# Autodesk Inventor assembly: Main Structure
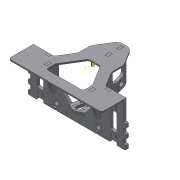
[picture p0: Inventor's stored thumbnail of the model, 180x180]
Saved by Autodesk Inventor 2015 (Build 190159000, 159)
## iProperties
Created: 2015-07-21
Part Number: Main Structure
Document SubType Name: Assembly
Designer: JR
Author: JR
## Documents named in this file (6)
- F:\OpenROV\2.8\Main Structure\Main Structure.iam
- F:\OpenROV\2.8\Main Structure\Bulkhead.ipt
- F:\OpenROV\2.8\Main Structure\Handle.ipt
- F:\OpenROV\2.8\Main Structure\Harness Pusher Final.ipt
- F:\OpenROV\2.8\Main Structure\Top Plate.ipt
- F:\OpenROV\2.8\Main Structure\Vert Moto Mount.ipt
## Components (6 placed, 5 different names)
1. Bulkhead:1 — Mate:1, Mate:2, Mate:3, Mate:7, Mate:8, Mate:9, Mate:10, Flush:1, Flush:2, Mate:11
2. Handle:1 — Mate:4, Mate:5, Mate:6, Mate:12, Mate:13
3. Harness Pusher Final:1 — Mate:8, Mate:9, Flush:2
4. Harness Pusher Final:2 — Mate:7, Mate:10, Flush:1
5. Top Plate:1 — Mate:11, Mate:12, Mate:13
6. Vert Moto Mount:1 — Mate:1, Mate:2, Mate:3, Mate:4, Mate:5, Mate:6
## Relationships (15: Mate 13, Flush 2)
- Mate:1: Bulkhead:1 ↔ Vert Moto Mount:1
- Mate:2: Bulkhead:1 ↔ Vert Moto Mount:1
- Mate:3: Bulkhead:1 ↔ Vert Moto Mount:1
- Mate:4: Handle:1 ↔ Vert Moto Mount:1
- Mate:5: Handle:1 ↔ Vert Moto Mount:1
- Mate:6: Handle:1 ↔ Vert Moto Mount:1
- Mate:7: Bulkhead:1 ↔ Harness Pusher Final:2
- Mate:8: Bulkhead:1 ↔ Harness Pusher Final:1
- Mate:9: Bulkhead:1 ↔ Harness Pusher Final:1
- Mate:10: Bulkhead:1 ↔ Harness Pusher Final:2
- Flush:1: Bulkhead:1 ↔ Harness Pusher Final:2
- Flush:2: Bulkhead:1 ↔ Harness Pusher Final:1
- Mate:11: Bulkhead:1 ↔ Top Plate:1
- Mate:12: Handle:1 ↔ Top Plate:1
- Mate:13: Handle:1 ↔ Top Plate:1
